# Autodesk Inventor assembly: A2017_T2_00
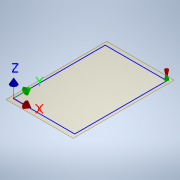
[picture p0: Inventor's stored thumbnail of the model, 180x180]
Saved by Autodesk Inventor 2022.3 (Build 263350000, 350)
## iProperties
Created: 2022-09-28
Part Number: A2017_T2_00
Document SubType Name: Assembly
Designer: Masato
Author: Masato
## Documents named in this file (2)
- C:\Users\Masato\Documents\EAGLE\projects\SUSTAINA-OP\Cam\A2017_T2\A2017_T2_00.iam
- C:\Users\Masato\Documents\EAGLE\projects\SUSTAINA-OP\Cam\DisposableBoard.ipt
## Components (1 placed, 1 different names)
1. DisposableBoard:1 — フラッシュ:1, フラッシュ:2, フラッシュ:3, フラッシュ:4
## Relationships (4: Flush 4)
- フラッシュ:1 [Flush]: DisposableBoard:1
- フラッシュ:2 [Flush]: DisposableBoard:1
- フラッシュ:3 [Flush]: DisposableBoard:1
- フラッシュ:4 [Flush]: DisposableBoard:1
